# Autodesk Inventor assembly: Objekt
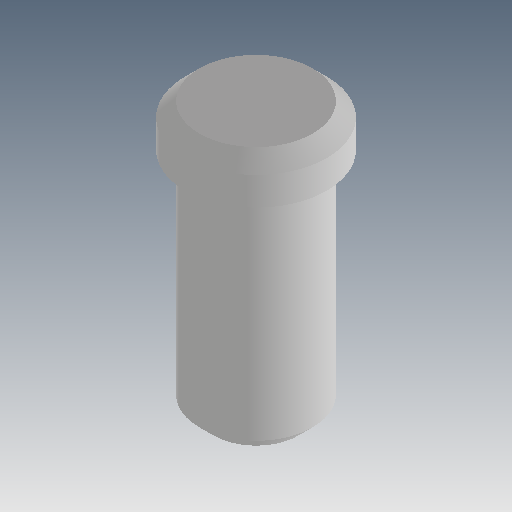
[picture p0: Inventor's stored thumbnail of the model, 512x512]
Saved by Autodesk Inventor 2020 (Build 240168000, 168)
## iProperties
Created: 2020-03-21
Part Number: Objekt
Document SubType Name: Assembly
Designer: franz
Author: franz
## Documents named in this file (3)
- E:\Privat\Projekte\SPS_Training\Unity_SPS_Simulation\Unity_SPS_Schrittkette\CAD\Foerderband_V1\Objekt\Objekt.iam
- E:\Privat\Projekte\SPS_Training\Unity_SPS_Simulation\Unity_SPS_Schrittkette\CAD\Foerderband_V1\Objekt\Dose_oben.ipt
- E:\Privat\Projekte\SPS_Training\Unity_SPS_Simulation\Unity_SPS_Schrittkette\CAD\Foerderband_V1\Objekt\Dose_unten.ipt
## Components (2 placed, 2 different names)
1. Dose_oben:1 — Starr:1
2. Dose_unten:1 — Starr:1
## Relationships (1: WeldJoint 1)
- Starr:1 [WeldJoint]: Dose_oben:1 ↔ Dose_unten:1
